# Autodesk Inventor assembly: GVS102 Housing
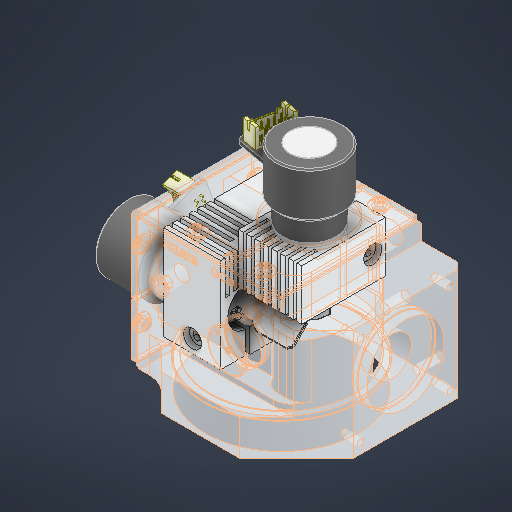
[picture p0: Inventor's stored thumbnail of the model, 512x512]
Saved by Autodesk Inventor 2025 (Build 290162000, 162)
## iProperties
Created: 2024-06-07
Part Number: GVS102 Housing
Document SubType Name: Assembly
Designer: mayhe
Author: mayhe
## Documents named in this file (3)
- C:\Users\mayhe\OneDrive\Documents\GitHub\In-situ-monitoring-of-powder-bed-fusion-additive-manufacturing\system_development\Orichalcum\v0.1\Hardware_design\galvo-scanner\GVS102 Housing.iam
- C:\Users\mayhe\OneDrive\Documents\GitHub\In-situ-monitoring-of-powder-bed-fusion-additive-manufacturing\system_development\Orichalcum\v0.2\Hardware_design\galvo-scanner\GVS102-Step.ipt
- C:\Users\mayhe\OneDrive\Documents\GitHub\In-situ-monitoring-of-powder-bed-fusion-additive-manufacturing\system_development\Orichalcum\v0.2\Hardware_design\galvo-scanner\GCM102_M-Step\GCM102_M-Step.ipt
## Components (2 placed, 2 different names)
1. GCM102_M-Step:1 — Mate:1
2. GVS102-Step:1 — Mate:1
## Relationships (1: Mate 1)
- Mate:1: GCM102_M-Step:1 ↔ GVS102-Step:1
